# Autodesk Inventor assembly: PT4
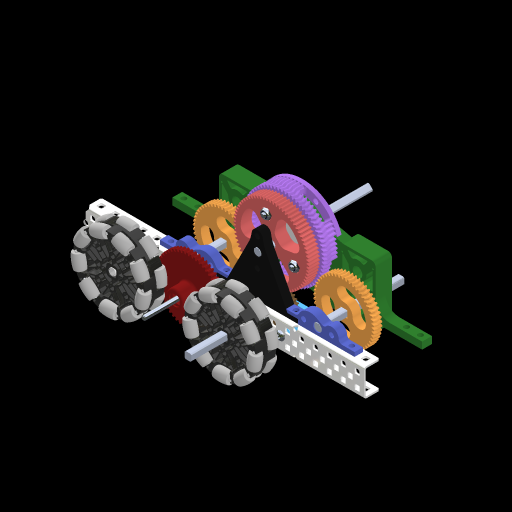
[picture p0: Inventor's stored thumbnail of the model, 512x512]
Saved by Autodesk Inventor 2024.1 (Build 281209000, 209)
## iProperties
Created: 2025-01-18
Part Number: PT4
Document SubType Name: Assembly
Designer: Teddy
Author: Teddy
## Documents named in this file (24)
- C:\Users\Teddy\OneDrive\Desktop\VEX-CAD-Inventor-1.4.0\pushBack\PushBackBot2\PT4.iam
- C:\Users\Teddy\OneDrive\Desktop\VEX-CAD-Inventor-1.4.0\2024-25 VexGame\GearBox\HerringBoneRingGear.ipt
- C:\Users\Teddy\OneDrive\Desktop\VEX-CAD-Inventor-1.4.0\2024-25 VexGame\GearBox\HerringBoneSunGear.ipt
- C:\Users\Teddy\OneDrive\Desktop\VEX-CAD-Inventor-1.4.0\2024-25 VexGame\GearBox\HerringBonePlanetGear.ipt
- C:\Users\Teddy\OneDrive\Desktop\VEX-CAD-Inventor-1.4.0\Structure\Hardware\Screw Steel - Star.ipt
- C:\Users\Teddy\OneDrive\Desktop\VEX-CAD-Inventor-1.4.0\Structure\Hardware\Nut Thin Nylock.ipt
- C:\Users\Teddy\OneDrive\Desktop\VEX-CAD-Inventor-1.4.0\2024-25 VexGame\GearBox\OffSetGear.ipt
- C:\Users\Teddy\OneDrive\Desktop\VEX-CAD-Inventor-1.4.0\Structure\Hardware\Screw Steel - Star\SScrew Star Smooth .875.ipt
- C:\Users\Teddy\OneDrive\Desktop\VEX-CAD-Inventor-1.4.0\Motion\Shaft HS\Shaft HS\Shaft HS 4.0 in.ipt
- C:\Users\Teddy\OneDrive\Desktop\VEX-CAD-Inventor-1.4.0\Motion\Shaft HS\Shaft HS.ipt
- C:\Users\Teddy\OneDrive\Desktop\VEX-CAD-Inventor-1.4.0\2024-25 VexGame\GearBox\HerringboneDriver.ipt
- C:\Users\Teddy\OneDrive\Desktop\VEX-CAD-Inventor-1.4.0\Structure\C Channel\Aluminum 1x2x1\Alu C 1x2x1x20.ipt
- C:\Users\Teddy\OneDrive\Desktop\VEX-CAD-Inventor-1.4.0\2024-25 VexGame\GearBox\OutPutGear.ipt
- C:\Users\Teddy\OneDrive\Desktop\VEX-CAD-Inventor-1.4.0\2024-25 VexGame\GearDriveTrain\TransmissonCoreMount.ipt
- C:\Users\Teddy\OneDrive\Desktop\VEX-CAD-Inventor-1.4.0\2024-25 VexGame\GearDriveTrain\DrivenMotorMount.ipt
- C:\Users\Teddy\OneDrive\Desktop\VEX-CAD-Inventor-1.4.0\2024-25 VexGame\GearDriveTrain\DrivenHolder.ipt
- C:\Users\Teddy\OneDrive\Desktop\VEX-CAD-Inventor-1.4.0\2024-25 VexGame\GearDriveTrain\MotorCapTransmission.ipt
- C:\Users\Teddy\OneDrive\Desktop\VEX-CAD-Inventor-1.4.0\Motion\Shaft HS\Shaft HS\Shaft HS 3.0 in.ipt
- C:\Users\Teddy\OneDrive\Desktop\VEX-CAD-Inventor-1.4.0\Motion\Shaft HS\Shaft HS\Shaft HS 3.5 in.ipt
- C:\Users\Teddy\OneDrive\Desktop\VEX-CAD-Inventor-1.4.0\Motion\Wheels\Omni Wheel\2.75 Omni AS, No Insert.iam
- C:\Users\Teddy\OneDrive\Desktop\VEX-CAD-Inventor-1.4.0\Motion\Wheels\Omni Wheel.iam
- C:\Users\Teddy\OneDrive\Desktop\VEX-CAD-Inventor-1.4.0\2024-25 VexGame\GearDriveTrain\GearTransmissionDTSmallAlternative.ipt
- C:\Users\Teddy\OneDrive\Desktop\VEX-CAD-Inventor-1.4.0\2024-25 VexGame\GearDriveTrain\GearTransmissionDTBig.ipt
- C:\Users\Teddy\OneDrive\Desktop\VEX-CAD-Inventor-1.4.0\Structure\Hardware\Screw Steel - Star\SScrew Star Smooth 2.000.ipt
## Components (35 placed, 20 different names)
1. HerringBoneRingGear:1
2. HerringBoneSunGear:1
3. HerringBonePlanetGear:1 — Insert:5, Insert:14
4. HerringBonePlanetGear:2 — Insert:6, Insert:11
5. HerringBonePlanetGear:3 — Insert:4, Insert:13
6. Nut Thin Nylock:1 — Insert:5, Insert:7
7. Nut Thin Nylock:2 — Insert:6
8. Nut Thin Nylock:3 — Insert:4
9. OffSetGear:1 — Insert:7, Insert:8, Insert:9, Insert:10, Insert:12
10. Nut Thin Nylock:4 — Insert:10
11. Nut Thin Nylock:5 — Insert:9
12. Nut Thin Nylock:6 — Insert:8
13. SScrew Star Smooth .875:1 — Insert:11
14. Shaft HS 4.0 in:1 — Insert:12, Insert:19
15. SScrew Star Smooth .875:2 — Insert:13
16. SScrew Star Smooth .875:3 — Insert:14
17. HerringboneDriver:1 — Insert:25, Insert:26
18. HerringboneDriver:2 — Insert:24, Insert:27
19. OutPutGear:1
20. TransmissonCoreMount:1 — Insert:19, Insert:21, Insert:23
21. DrivenMotorMount:1 — Insert:21, Insert:24, Insert:30
22. DrivenMotorMount:2 — Insert:23, Insert:25, Insert:31
23. DrivenHolder:1 — Insert:32
24. MotorCapTransmission:1 — Insert:26, Insert:27
25. Alu C 1x2x1x20:1 — Insert:35, Insert:36, Insert:37, Insert:39, Insert:40
26. Shaft HS 3.0 in:2 — Insert:30
27. Shaft HS 3.0 in:3 — Insert:31
28. Shaft HS 3.5 in:4 — Insert:32
29. 2.75 Omni AS, No Insert:1 [sub-assembly] — Insert:33, Insert:34
30. 2.75 Omni AS, No Insert:2 [sub-assembly] — Insert:38
31. GearTransmissionDTSmallAlternative:1 — Insert:37, Insert:38
32. GearTransmissionDTSmallAlternative:2 — Insert:33, Insert:34, Insert:35
33. GearTransmissionDTBig:1 — Insert:36
34. SScrew Star Smooth 2.000:4 — Insert:39
35. SScrew Star Smooth 2.000:6 — Insert:40
## Relationships (29: Insert 29)
- Insert:4: HerringBonePlanetGear:3 ↔ Nut Thin Nylock:3
- Insert:5: HerringBonePlanetGear:1 ↔ Nut Thin Nylock:1
- Insert:6: HerringBonePlanetGear:2 ↔ Nut Thin Nylock:2
- Insert:7: Nut Thin Nylock:1 ↔ OffSetGear:1
- Insert:8: OffSetGear:1 ↔ Nut Thin Nylock:6
- Insert:9: OffSetGear:1 ↔ Nut Thin Nylock:5
- Insert:10: OffSetGear:1 ↔ Nut Thin Nylock:4
- Insert:11: HerringBonePlanetGear:2 ↔ SScrew Star Smooth .875:1
- Insert:12 (-12.7 mm): OffSetGear:1 ↔ Shaft HS 4.0 in:1
- Insert:13: HerringBonePlanetGear:3 ↔ SScrew Star Smooth .875:2
- Insert:14: HerringBonePlanetGear:1 ↔ SScrew Star Smooth .875:3
- Insert:19: Shaft HS 4.0 in:1 ↔ TransmissonCoreMount:1
- Insert:21: TransmissonCoreMount:1 ↔ DrivenMotorMount:1
- Insert:23: TransmissonCoreMount:1 ↔ DrivenMotorMount:2
- Insert:24 (16.256 mm): HerringboneDriver:2 ↔ DrivenMotorMount:1
- Insert:25 (16.256 mm): HerringboneDriver:1 ↔ DrivenMotorMount:2
- Insert:26 (5.08 mm): HerringboneDriver:1 ↔ MotorCapTransmission:1
- Insert:27 (5.08 mm): HerringboneDriver:2 ↔ MotorCapTransmission:1
- Insert:30: DrivenMotorMount:1 ↔ Shaft HS 3.0 in:2
- Insert:31: DrivenMotorMount:2 ↔ Shaft HS 3.0 in:3
- Insert:32: DrivenHolder:1 ↔ Shaft HS 3.5 in:4
- Insert:33: 2.75 Omni AS, No Insert:1 ↔ GearTransmissionDTSmallAlternative:2
- Insert:34: 2.75 Omni AS, No Insert:1 ↔ GearTransmissionDTSmallAlternative:2
- Insert:35 (2.54 mm): Alu C 1x2x1x20:1 ↔ GearTransmissionDTSmallAlternative:2
- Insert:36 (2.54 mm): Alu C 1x2x1x20:1 ↔ GearTransmissionDTBig:1
- Insert:37 (2.54 mm): Alu C 1x2x1x20:1 ↔ GearTransmissionDTSmallAlternative:1
- Insert:38: 2.75 Omni AS, No Insert:2 ↔ GearTransmissionDTSmallAlternative:1
- Insert:39: Alu C 1x2x1x20:1 ↔ SScrew Star Smooth 2.000:4
- Insert:40: Alu C 1x2x1x20:1 ↔ SScrew Star Smooth 2.000:6
